# Autodesk Inventor assembly: Zynq_Z010_uZed_F_Prod
(part 2 of 2)
209. 861 [sub-assembly]
210. 865 [sub-assembly]
211. 869 [sub-assembly]
212. 873 [sub-assembly]
213. 877 [sub-assembly]
214. 881 [sub-assembly]
215. 887 [sub-assembly]
216. 891 [sub-assembly]
217. 895 [sub-assembly]
218. 900 [sub-assembly]
219. 908 [sub-assembly]
220. 917 [sub-assembly]
221. 921 [sub-assembly]
222. 925 [sub-assembly]
223. 931 [sub-assembly]
224. 939 [sub-assembly]
225. 944 [sub-assembly]
226. 948 [sub-assembly]
227. 996 [sub-assembly]
228. 1051 [sub-assembly]
229. 1055 [sub-assembly]
230. 1062 [sub-assembly]
231. 1067 [sub-assembly]
232. 1072 [sub-assembly]
233. 1074 [sub-assembly]
234. 1076 [sub-assembly]
235. 1082 [sub-assembly]
236. 1088 [sub-assembly]
237. 1092 [sub-assembly]
238. 1096 [sub-assembly]
239. 1100 [sub-assembly]
240. 1105 [sub-assembly]
241. 1109 [sub-assembly]
242. 1113 [sub-assembly]
243. 1120 [sub-assembly]
244. 1124 [sub-assembly]
245. 1128 [sub-assembly]
246. 1132 [sub-assembly]
247. 1136 [sub-assembly]
248. 1140 [sub-assembly]
249. 1144 [sub-assembly]
250. 1148 [sub-assembly]
251. 1152 [sub-assembly]
252. 1156 [sub-assembly]
253. 1160 [sub-assembly]
254. 1164 [sub-assembly]
255. 1168 [sub-assembly]
256. 1172 [sub-assembly]
257. 1176 [sub-assembly]
258. 1180 [sub-assembly]
259. 1184 [sub-assembly]
260. 1188 [sub-assembly]
261. 1192 [sub-assembly]
262. 1196 [sub-assembly]
263. 1200 [sub-assembly]
264. 1204 [sub-assembly]
265. 1208 [sub-assembly]
266. 1212 [sub-assembly]
267. 1216 [sub-assembly]
268. 1220 [sub-assembly]
269. 1224 [sub-assembly]
270. 1228 [sub-assembly]
271. 1232 [sub-assembly]
272. 1236 [sub-assembly]
273. 1240 [sub-assembly]
274. 1244 [sub-assembly]
275. 1248 [sub-assembly]
276. 1252 [sub-assembly]
277. 1256 [sub-assembly]
278. 1260 [sub-assembly]
279. 1264 [sub-assembly]
280. 1268 [sub-assembly]
281. 1272 [sub-assembly]
282. 1276 [sub-assembly]
283. 1280 [sub-assembly]
284. 1284 [sub-assembly]
285. 1288 [sub-assembly]
286. 1292 [sub-assembly]
287. 1296 [sub-assembly]
288. 1300 [sub-assembly]
289. 1304 [sub-assembly]
290. 1308 [sub-assembly]
291. 1312 [sub-assembly]
292. 1318 [sub-assembly]
293. 1322 [sub-assembly]
294. 1326 [sub-assembly]
295. 1330 [sub-assembly]
296. 1334 [sub-assembly]
297. 1338 [sub-assembly]
298. 1342 [sub-assembly]
299. 1346 [sub-assembly]
300. 1350 [sub-assembly]
301. 1354 [sub-assembly]
302. 1358 [sub-assembly]
303. 1362 [sub-assembly]
304. 1366 [sub-assembly]
305. 1370 [sub-assembly]
306. 1374 [sub-assembly]
307. 1378 [sub-assembly]
308. 1382 [sub-assembly]
309. 1386 [sub-assembly]
310. 1390 [sub-assembly]
311. 1394 [sub-assembly]
312. 1398 [sub-assembly]
313. 1402 [sub-assembly]
314. 1406 [sub-assembly]
315. 1410 [sub-assembly]
316. 1414 [sub-assembly]
317. 1418 [sub-assembly]
318. 1422 [sub-assembly]
319. 1426 [sub-assembly]
320. 1430 [sub-assembly]
321. 1434 [sub-assembly]
322. 1438 [sub-assembly]
323. 1450 [sub-assembly]
324. 1462 [sub-assembly]
325. 1467 [sub-assembly]
326. 1470 [sub-assembly]
327. 1475 [sub-assembly]
328. 1478 [sub-assembly]
329. 1482 [sub-assembly]
330. 1487 [sub-assembly]
331. 1492 [sub-assembly]
332. 1497 [sub-assembly]
333. 1506 [sub-assembly]
334. 1511 [sub-assembly]
335. 1516 [sub-assembly]
336. 1521 [sub-assembly]
337. 1524 [sub-assembly]
338. 1527 [sub-assembly]
339. 1530 [sub-assembly]
340. 1545 [sub-assembly]
341. 1558 [sub-assembly]
342. 1569 [sub-assembly]
343. 1575 [sub-assembly]
344. 1581 [sub-assembly]
345. 1586 [sub-assembly]
346. 1591 [sub-assembly]
347. 1594 [sub-assembly]
348. 1597 [sub-assembly]
349. 1600 [sub-assembly]
350. 1604 [sub-assembly]
351. 1608 [sub-assembly]
352. 1612 [sub-assembly]
353. 1616 [sub-assembly]
354. 1623 [sub-assembly]
355. 1628 [sub-assembly]
356. 1633 [sub-assembly]
357. 1638 [sub-assembly]
358. 1642 [sub-assembly]
359. 1647 [sub-assembly]
360. 1652 [sub-assembly]
